# Autodesk Inventor assembly: CollectorAssemblyGB
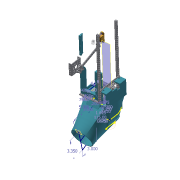
[picture p0: Inventor's stored thumbnail of the model, 180x180]
Saved by Autodesk Inventor 2018 (Build 220112000, 112)
## iProperties
Created: 2018-10-28
Part Number: CollectorAssemblyGB
Document SubType Name: Assembly
Designer: ball
Author: ball
## Documents named in this file (28)
- C:\FTC\FTC8863CAD\2018Robot\CollectorAssemblyWithChute.iam
- C:\FTC\FTC8863CAD\GoBilda\1103 Parts\1106-0035-0280.ipt
- C:\FTC\FTC8863CAD\GoBilda\1121 Parts\1121-0011-0288.ipt
- C:\FTC\FTC8863CAD\2018Robot\ServoWithPlateCoupler.iam
- C:\FTC\FTC8863CAD\GoBilda\1501 Parts\1501-0006-0240.ipt
- C:\FTC\FTC8863CAD\GoBilda\2905 Parts\2905-0006-0008 assembly.ipt
- C:\FTC\FTC8863CAD\GoBilda\1601 Parts\1601-0014-0006.ipt
- C:\FTC\FTC8863CAD\GoBilda\2101 Parts\2101-0006-0090.ipt
- C:\FTC\FTC8863CAD\Andymark\am-0619a+Entrapption+Star,+4.75+Diameter.ipt
- C:\FTC\FTC8863CAD\Andymark\am-2850+wiffle+base+Ball.ipt
- C:\FTC\FTC8863CAD\GoBilda\1103 Parts\1103-0011-0088.ipt
- C:\FTC\FTC8863CAD\GoBilda\1121 Parts\1121-0007-0192.ipt
- C:\FTC\FTC8863CAD\RevRobotics\REV-31-1537.ipt
- C:\FTC\FTC8863CAD\GoBilda\1121 Parts\1121-0001-0048.ipt
- C:\FTC\FTC8863CAD\GoBilda\2101 Parts\2101-0006-0080.ipt
- C:\FTC\FTC8863CAD\2018Robot\SensorWall.ipt
- C:\FTC\FTC8863CAD\GoBilda\1301 Parts\1301-0016-0006 assembly.ipt
- C:\FTC\FTC8863CAD\2018Robot\MineralStop1.00x75WithCuts.ipt
- C:\FTC\FTC8863CAD\2018Robot\ChuteRoof.ipt
- C:\FTC\FTC8863CAD\2018Robot\EjectionRamp.ipt
- C:\FTC\FTC8863CAD\2018Robot\Back Wall.ipt
- C:\FTC\FTC8863CAD\2018Robot\Flat Roof panel.ipt
- C:\FTC\FTC8863CAD\2018Robot\CollectorArm165.ipt
- C:\FTC\FTC8863CAD\2018Robot\CollectorArmRear5_0.ipt
- C:\FTC\FTC8863CAD\GoBilda\1103 Parts\1103-0013-0104.ipt
- C:\FTC\FTC8863CAD\2018Robot\CollectorChute25degreesNoMotorCutout.ipt
- C:\FTC\FTC8863CAD\2018Robot\CollectorChute25DegreesRoof.ipt
- C:\FTC\FTC8863CAD\StepLibraries\Screws\M4x12 SS PAN HEAD PHIL MACHINE SCREW.ipt
## Components (44 placed, 27 different names)
1. 1106-0035-0280:1 — Flush:1, Flush:2, Flush:4, Mate:62, Mate:63, Flush:5, Mate:70, Mate:100, Mate:105, Mate:108, Symmetry:2, Mate:123
2. 1106-0035-0280:2 — Flush:1, Flush:4, Mate:13, Mate:57, Mate:59, Mate:69, Mate:90, Mate:91, Mate:92, Symmetry:1, Symmetry:2, Flush:29, Mate:116, Mate:122, Flush:32
3. 1106-0035-0280:3 — Flush:2, Mate:58, Mate:69, Mate:74, Mate:75, Mate:93, Mate:95, Angle:3, Symmetry:1, Flush:28
4. 1106-0035-0280:4 — Mate:61, Flush:5, Mate:64, Mate:70, Angle:2
5. 1121-0011-0288:1 — Mate:13, Mate:22, Mate:23, Mate:24, Mate:25, Mate:26, Mate:27, Mate:37, Mate:38, Mate:68
6. ServoWithPlateCoupler:1 [sub-assembly] — Mate:15, Mate:17, Mate:19, Mate:21, Mate:22, Mate:27
7. 1501-0006-0240:2 — Mate:15, Mate:23
8. 1501-0006-0240:3 — Mate:19, Mate:25
9. 1501-0006-0240:4 — Mate:17, Mate:26
10. 1501-0006-0240:5 — Mate:21, Mate:24
11. 2905-0006-0008 assembly:1 — Mate:42, Mate:43
12. 2905-0006-0008 assembly:2 — Mate:44, Mate:45
13. 1601-0014-0006:1 — Mate:41, Mate:42, Mate:66
14. 1601-0014-0006:2 — Mate:37, Mate:38, Mate:40, Mate:44
15. 2101-0006-0090:1 — Mate:40, Mate:41, Mate:43, Mate:45, Mate:65, Mate:66, Mate:67
16. am-0619a+Entrapption+Star,+4.75+Diameter:1 — Mate:67, Mate:97, Flush:13
17. am-0619a+Entrapption+Star,+4.75+Diameter:2 — Mate:68, Mate:98
18. am-2850+wiffle+base+Ball:1
19. 1103-0011-0088:2 — Mate:61, Mate:62, Mate:63, Mate:107
20. 1103-0011-0088:3 — Mate:57, Mate:58, Mate:59, Mate:106, Flush:17, Mate:115, Mate:119, Mate:120, Mate:121
21. 1121-0007-0192:2 — Mate:64, Mate:65, Mate:74, Mate:75, Mate:97, Mate:98
22. REV-31-1537:3 — Angle:2, Mate:103, Mate:104
23. ServoWithPlateCoupler:2 [sub-assembly] — Mate:88, Mate:89, Angle:1, Flush:8
24. 1501-0006-0240:6 — Mate:83, Mate:86
25. 1501-0006-0240:7 — Mate:84
26. 1501-0006-0240:8 — Mate:85
27. 1501-0006-0240:9 — Mate:88
28. 1121-0001-0048:1 — Mate:83, Mate:84, Mate:85, Mate:86, Mate:89, Angle:1, Mate:90, Mate:91, Mate:92, Mate:94, Flush:7
29. 1121-0001-0048:2 — Mate:93, Mate:94, Flush:7, Mate:95
30. 2101-0006-0080:2 — Flush:8, Mate:99
31. SensorWall:1 — Mate:100, Mate:103, Mate:104, Mate:105, Mate:108
32. 1301-0016-0006 assembly:1 — Mate:99, Flush:13, Flush:14, Mate:109, Mate:110, Mate:111, Mate:113, Mate:114
33. MineralStop1.00x75WithCuts:1 — Mate:106, Mate:107, Flush:17, Mate:115
34. ChuteRoof:1 — Flush:26
35. EjectionRamp:1 — Flush:28
36. Back Wall:1 — Flush:29
37. Flat Roof panel:1
38. CollectorArm165:1 — Mate:109, Mate:110, Mate:111, Mate:112
39. CollectorArmRear5_0:1 — Mate:112, Mate:113, Mate:114
40. 1103-0013-0104:1 — Mate:116, Mate:122, Mate:123, Flush:30, Mate:124, Mate:125, Mate:126, Mate:127
41. CollectorChute25degreesNoMotorCutout:1 — Mate:119, Mate:120, Mate:121, Flush:33, Flush:34, Flush:35
42. CollectorChute25DegreesRoof:1 — Flush:30, Flush:32, Flush:33, Flush:34, Flush:35
43. M4x12 SS PAN HEAD PHIL MACHINE SCREW:1 — Mate:124, Mate:127
44. M4x12 SS PAN HEAD PHIL MACHINE SCREW:2 — Mate:125, Mate:126
## Relationships (100: Mate 78, Flush 17, Angle 3, Symmetry 2)
- Flush:1: 1106-0035-0280:1 ↔ 1106-0035-0280:2
- Flush:2: 1106-0035-0280:1 ↔ 1106-0035-0280:3
- Flush:4: 1106-0035-0280:1 ↔ 1106-0035-0280:2
- Mate:13: 1106-0035-0280:2 ↔ 1121-0011-0288:1
- Mate:15: ServoWithPlateCoupler:1 ↔ 1501-0006-0240:2
- Mate:17: ServoWithPlateCoupler:1 ↔ 1501-0006-0240:4
- Mate:19: ServoWithPlateCoupler:1 ↔ 1501-0006-0240:3
- Mate:21: ServoWithPlateCoupler:1 ↔ 1501-0006-0240:5
- Mate:22: 1121-0011-0288:1 ↔ ServoWithPlateCoupler:1
- Mate:23: 1121-0011-0288:1 ↔ 1501-0006-0240:2
- Mate:24: 1121-0011-0288:1 ↔ 1501-0006-0240:5
- Mate:25: 1121-0011-0288:1 ↔ 1501-0006-0240:3
- Mate:26: 1121-0011-0288:1 ↔ 1501-0006-0240:4
- Mate:27 (24 mm): 1121-0011-0288:1 ↔ ServoWithPlateCoupler:1
- Mate:37: 1121-0011-0288:1 ↔ 1601-0014-0006:2
- Mate:38: 1121-0011-0288:1 ↔ 1601-0014-0006:2
- Mate:40: 1601-0014-0006:2 ↔ 2101-0006-0090:1
- Mate:41: 1601-0014-0006:1 ↔ 2101-0006-0090:1
- Mate:42: 2905-0006-0008 assembly:1 ↔ 1601-0014-0006:1
- Mate:43: 2905-0006-0008 assembly:1 ↔ 2101-0006-0090:1
- Mate:44: 2905-0006-0008 assembly:2 ↔ 1601-0014-0006:2
- Mate:45: 2905-0006-0008 assembly:2 ↔ 2101-0006-0090:1
- Mate:57: 1106-0035-0280:2 ↔ 1103-0011-0088:3
- Mate:58: 1106-0035-0280:3 ↔ 1103-0011-0088:3
- Mate:59: 1106-0035-0280:2 ↔ 1103-0011-0088:3
- Mate:61: 1106-0035-0280:4 ↔ 1103-0011-0088:2
- Mate:62: 1106-0035-0280:1 ↔ 1103-0011-0088:2
- Mate:63: 1106-0035-0280:1 ↔ 1103-0011-0088:2
- Flush:5: 1106-0035-0280:1 ↔ 1106-0035-0280:4
- Mate:64: 1106-0035-0280:4 ↔ 1121-0007-0192:2
- Mate:65: 2101-0006-0090:1 ↔ 1121-0007-0192:2
- Mate:66: 1601-0014-0006:1 ↔ 2101-0006-0090:1
- Mate:67: 2101-0006-0090:1 ↔ am-0619a+Entrapption+Star,+4.75+Diameter:1
- Mate:68: 1121-0011-0288:1 ↔ am-0619a+Entrapption+Star,+4.75+Diameter:2
- Mate:69: 1106-0035-0280:2 ↔ 1106-0035-0280:3
- Mate:70: 1106-0035-0280:1 ↔ 1106-0035-0280:4
- Mate:74: 1106-0035-0280:3 ↔ 1121-0007-0192:2
- Mate:75: 1106-0035-0280:3 ↔ 1121-0007-0192:2
- [Mate]: ServoWithPlateCoupler:2 ↔ 1501-0006-0240:6
- [Mate]: ServoWithPlateCoupler:2 ↔ 1501-0006-0240:8
- [Mate]: ServoWithPlateCoupler:2 ↔ 1501-0006-0240:7
- [Mate]: ServoWithPlateCoupler:2 ↔ 1501-0006-0240:9
- Mate:83: 1501-0006-0240:6 ↔ 1121-0001-0048:1
- Mate:84: 1501-0006-0240:7 ↔ 1121-0001-0048:1
- Mate:85: 1501-0006-0240:8 ↔ 1121-0001-0048:1
- Mate:86: 1501-0006-0240:6 ↔ 1121-0001-0048:1
- Mate:88: ServoWithPlateCoupler:2 ↔ 1501-0006-0240:9
- Mate:89: ServoWithPlateCoupler:2 ↔ 1121-0001-0048:1
- Angle:1 (0 deg): ServoWithPlateCoupler:2 ↔ 1121-0001-0048:1
- Mate:90: 1106-0035-0280:2 ↔ 1121-0001-0048:1
- Mate:91: 1106-0035-0280:2 ↔ 1121-0001-0048:1
- Mate:92: 1106-0035-0280:2 ↔ 1121-0001-0048:1
- Mate:93: 1106-0035-0280:3 ↔ 1121-0001-0048:2
- Mate:94: 1121-0001-0048:1 ↔ 1121-0001-0048:2
- Flush:7: 1121-0001-0048:1 ↔ 1121-0001-0048:2
- Mate:95: 1106-0035-0280:3 ↔ 1121-0001-0048:2
- [Mate]: 1121-0001-0048:2 ↔ 2101-0006-0080:2
- Flush:8: ServoWithPlateCoupler:2 ↔ 2101-0006-0080:2
- Mate:97 (33.3375 mm): am-0619a+Entrapption+Star,+4.75+Diameter:1 ↔ 1121-0007-0192:2
- Mate:98 (19.05 mm): am-0619a+Entrapption+Star,+4.75+Diameter:2 ↔ 1121-0007-0192:2
- Angle:2 (0 deg): 1106-0035-0280:4 ↔ REV-31-1537:3
- Mate:99: 2101-0006-0080:2 ↔ 1301-0016-0006 assembly:1
- Flush:13 (-6.35 mm): am-0619a+Entrapption+Star,+4.75+Diameter:1 ↔ 1301-0016-0006 assembly:1
- Flush:14 (-7.0104 mm): 1301-0016-0006 assembly:1
- Angle:3 (18.3 deg): 1106-0035-0280:3
- Mate:100: 1106-0035-0280:1 ↔ SensorWall:1
- Mate:103: REV-31-1537:3 ↔ SensorWall:1
- Mate:104: REV-31-1537:3 ↔ SensorWall:1
- Mate:105: 1106-0035-0280:1 ↔ SensorWall:1
- Mate:106: 1103-0011-0088:3 ↔ MineralStop1.00x75WithCuts:1
- Mate:107: 1103-0011-0088:2 ↔ MineralStop1.00x75WithCuts:1
- Flush:17: 1103-0011-0088:3 ↔ MineralStop1.00x75WithCuts:1
- Mate:108: 1106-0035-0280:1 ↔ SensorWall:1
- Symmetry:1: 1106-0035-0280:2 ↔ 1106-0035-0280:3
- Symmetry:2: 1106-0035-0280:1 ↔ 1106-0035-0280:2
- Flush:26: ChuteRoof:1
- Flush:28: 1106-0035-0280:3 ↔ EjectionRamp:1
- Flush:29: 1106-0035-0280:2 ↔ Back Wall:1
- Mate:109: 1301-0016-0006 assembly:1 ↔ CollectorArm165:1
- Mate:110: 1301-0016-0006 assembly:1 ↔ CollectorArm165:1
- Mate:111: 1301-0016-0006 assembly:1 ↔ CollectorArm165:1
- Mate:112: CollectorArm165:1 ↔ CollectorArmRear5_0:1
- Mate:113: 1301-0016-0006 assembly:1 ↔ CollectorArmRear5_0:1
- Mate:114: 1301-0016-0006 assembly:1 ↔ CollectorArmRear5_0:1
- Mate:115: 1103-0011-0088:3 ↔ MineralStop1.00x75WithCuts:1
- Mate:116: 1106-0035-0280:2 ↔ 1103-0013-0104:1
- Mate:119: 1103-0011-0088:3 ↔ CollectorChute25degreesNoMotorCutout:1
- Mate:120: 1103-0011-0088:3 ↔ CollectorChute25degreesNoMotorCutout:1
- Mate:121: 1103-0011-0088:3 ↔ CollectorChute25degreesNoMotorCutout:1
- Mate:122: 1106-0035-0280:2 ↔ 1103-0013-0104:1
- Mate:123: 1106-0035-0280:1 ↔ 1103-0013-0104:1
- Flush:30: 1103-0013-0104:1 ↔ CollectorChute25DegreesRoof:1
- Flush:32: 1106-0035-0280:2 ↔ CollectorChute25DegreesRoof:1
- Flush:33: CollectorChute25degreesNoMotorCutout:1 ↔ CollectorChute25DegreesRoof:1
- Flush:34: CollectorChute25degreesNoMotorCutout:1 ↔ CollectorChute25DegreesRoof:1
- Flush:35: CollectorChute25degreesNoMotorCutout:1 ↔ CollectorChute25DegreesRoof:1
- Mate:124: 1103-0013-0104:1 ↔ M4x12 SS PAN HEAD PHIL MACHINE SCREW:1
- Mate:125: 1103-0013-0104:1 ↔ M4x12 SS PAN HEAD PHIL MACHINE SCREW:2
- Mate:126: 1103-0013-0104:1 ↔ M4x12 SS PAN HEAD PHIL MACHINE SCREW:2
- Mate:127: 1103-0013-0104:1 ↔ M4x12 SS PAN HEAD PHIL MACHINE SCREW:1
## Named parameters: d97_d28 = 0 mm, d98_d30 = 0 mm, d99_d32 = 0 mm, d100_d34 = 0 mm
